# Autodesk Inventor assembly: Vỏ máy
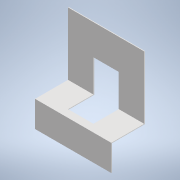
[picture p0: Inventor's stored thumbnail of the model, 180x180]
Saved by Autodesk Inventor 2020 (Build 240168000, 168)
## iProperties
Created: 2022-11-30
Part Number: Vỏ máy
Document SubType Name: Assembly
Designer: ADMIN
Author: ADMIN
## Documents named in this file (4)
- D:\Do-an-tot-nghiep\Inventor\Vỏ máy.iam
- D:\Do-an-tot-nghiep\Inventor\Vỏ U1.ipt
- D:\Do-an-tot-nghiep\Inventor\Vỏ F1.ipt
- D:\Do-an-tot-nghiep\Inventor\Vỏ F2.ipt
## Components (3 placed, 3 different names)
1. Vỏ U1:1 — Flush:1, Mate:1, Flush:2, Flush:3, Mate:2, Flush:4
2. Vỏ F1:1 — Flush:1, Mate:1, Flush:2
3. Vỏ F2:1 — Flush:3, Mate:2, Flush:4
## Relationships (6: Flush 4, Mate 2)
- Flush:1: Vỏ U1:1 ↔ Vỏ F1:1
- Mate:1: Vỏ U1:1 ↔ Vỏ F1:1
- Flush:2: Vỏ U1:1 ↔ Vỏ F1:1
- Flush:3: Vỏ U1:1 ↔ Vỏ F2:1
- Mate:2: Vỏ U1:1 ↔ Vỏ F2:1
- Flush:4: Vỏ U1:1 ↔ Vỏ F2:1
